# Autodesk Inventor assembly: Main Assembly
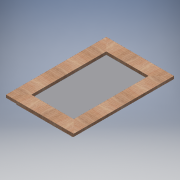
[picture p0: Inventor's stored thumbnail of the model, 180x180]
Saved by Autodesk Inventor 2017 (Build 210142000, 142)
## iProperties
Created: 2019-02-16
Part Number: Main Assembly
Document SubType Name: Assembly
Designer: Mitch
Author: Mitch
## Documents named in this file (7)
- E:\Youtube Channel\Pojects\Magic Mirror\Main Assembly.iam
- E:\Youtube Channel\Pojects\Magic Mirror\LCD Screen.ipt
- E:\Youtube Channel\Pojects\Magic Mirror\TopnBottom Border.ipt
- E:\Youtube Channel\Pojects\Magic Mirror\Side Border.ipt
- E:\Youtube Channel\Pojects\Magic Mirror\side box.ipt
- E:\Youtube Channel\Pojects\Magic Mirror\topnbottom box.ipt
- E:\Youtube Channel\Pojects\Magic Mirror\bracket.ipt
## Components (13 placed, 6 different names)
1. LCD Screen:1 — Mate:7, Mate:8, Mate:9
2. TopnBottom Border:1 — Mate:1, Flush:1, Mate:2, Mate:3, Flush:2, Mate:4, Mate:8, Flush:5, Flush:7, Mate:15, Mate:21
3. TopnBottom Border:2 — Mate:5, Flush:3, Mate:6, Mate:13, Mate:16, Mate:19
4. Side Border:1 — Mate:1, Flush:1, Mate:2, Mate:5, Flush:3, Mate:6, Flush:6, Mate:11
5. Side Border:2 — Mate:3, Flush:2, Mate:4, Mate:7, Mate:9, Flush:4, Mate:10, Mate:20
6. side box:1 — Flush:6, Mate:11, Flush:7, Mate:12, Flush:8, Mate:22, Mate:26
7. side box:2 — Flush:4, Mate:10, Flush:5, Mate:14, Flush:9, Mate:17, Mate:24
8. topnbottom box:1 — Mate:12, Mate:13, Flush:8, Mate:18, Mate:23
9. topnbottom box:2 — Mate:14, Mate:15, Flush:9, Mate:25, Mate:27
10. bracket:1 — Mate:16, Mate:17, Mate:18
11. bracket:2 — Mate:19, Mate:26, Mate:27
12. bracket:3 — Mate:20, Mate:22, Mate:23
13. bracket:4 — Mate:21, Mate:24, Mate:25
## Relationships (36: Mate 27, Flush 9)
- Mate:1: TopnBottom Border:1 ↔ Side Border:1
- Flush:1: TopnBottom Border:1 ↔ Side Border:1
- Mate:2: TopnBottom Border:1 ↔ Side Border:1
- Mate:3: TopnBottom Border:1 ↔ Side Border:2
- Flush:2: TopnBottom Border:1 ↔ Side Border:2
- Mate:4: TopnBottom Border:1 ↔ Side Border:2
- Mate:5: TopnBottom Border:2 ↔ Side Border:1
- Flush:3: TopnBottom Border:2 ↔ Side Border:1
- Mate:6: TopnBottom Border:2 ↔ Side Border:1
- Mate:7: LCD Screen:1 ↔ Side Border:2
- Mate:8: LCD Screen:1 ↔ TopnBottom Border:1
- Mate:9: LCD Screen:1 ↔ Side Border:2
- Flush:4 (38.989 mm): Side Border:2 ↔ side box:2
- Mate:10: Side Border:2 ↔ side box:2
- Flush:5 (44.45 mm): TopnBottom Border:1 ↔ side box:2
- Flush:6 (38.989 mm): Side Border:1 ↔ side box:1
- Mate:11: Side Border:1 ↔ side box:1
- Flush:7 (44.45 mm): TopnBottom Border:1 ↔ side box:1
- Mate:12: side box:1 ↔ topnbottom box:1
- Mate:13: TopnBottom Border:2 ↔ topnbottom box:1
- Flush:8: side box:1 ↔ topnbottom box:1
- Mate:14: side box:2 ↔ topnbottom box:2
- Mate:15: TopnBottom Border:1 ↔ topnbottom box:2
- Flush:9: side box:2 ↔ topnbottom box:2
- Mate:16: TopnBottom Border:2 ↔ bracket:1
- Mate:17: side box:2 ↔ bracket:1
- Mate:18: topnbottom box:1 ↔ bracket:1
- Mate:19: TopnBottom Border:2 ↔ bracket:2
- Mate:20: Side Border:2 ↔ bracket:3
- Mate:21: TopnBottom Border:1 ↔ bracket:4
- Mate:22: side box:1 ↔ bracket:3
- Mate:23: topnbottom box:1 ↔ bracket:3
- Mate:24: side box:2 ↔ bracket:4
- Mate:25: topnbottom box:2 ↔ bracket:4
- Mate:26: side box:1 ↔ bracket:2
- Mate:27: topnbottom box:2 ↔ bracket:2
